# Autodesk Inventor assembly: Galileo Extruder
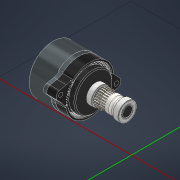
[picture p0: Inventor's stored thumbnail of the model, 180x180]
Saved by Autodesk Inventor 2022.2 (Build 262287010, 287A)
## iProperties
Created: 2022-03-15
Part Number: Galileo Extruder
Document SubType Name: Assembly
Designer: sleib
Author: sleib
## Documents named in this file (7)
- C:\Users\sleib\Projekte\Voron-2\CAD\Inventor\Galileo Clockwork\Galileo Extruder.iam
- C:\Users\sleib\Projekte\Voron-2\CAD\Inventor\Galileo Clockwork\Spacer Shim.ipt
- C:\Users\sleib\Projekte\Voron-2\CAD\Inventor\Galileo Clockwork\Updated Gearset MJF Shaft + Carrier.iam
- C:\Users\sleib\Projekte\Voron-2\CAD\Inventor\Galileo Clockwork\MotorGear.ipt
- C:\Users\sleib\Projekte\Voron-2\CAD\Inventor\Galileo Clockwork\Ring Gear Housing.ipt
- C:\Users\sleib\Projekte\Voron-2\CAD\Inventor\Galileo Clockwork\Stepper Body.ipt
- C:\Users\sleib\Projekte\Voron-2\CAD\Inventor\Galileo Clockwork\MR148ZZ v1.iam
## Components (7 placed, 6 different names)
1. Stepper Body:1 — Passend:17, Fluchtend:1, Passend:18, Passend:19, Passend:20, Fluchtend:2, Passend:21
2. Spacer Shim:1 — Passend:3, Passend:16, Passend:24
3. Updated Gearset MJF Shaft + Carrier:1 [sub-assembly] — Passend:3, Passend:15, Passend:20, Fluchtend:2, Passend:22, Passend:23, Fluchtend:3
4. MotorGear:1 — Passend:15, Passend:16, Passend:25
5. Ring Gear Housing:1 — Passend:18, Passend:19, Passend:21
6. MR148ZZ v1:1 [sub-assembly] — Passend:22, Passend:24
7. MR148ZZ v1:2 [sub-assembly] — Passend:23, Passend:25, Fluchtend:3
## Relationships (15: Mate 12, Flush 3)
- Passend:3 [Mate]: Spacer Shim:1 ↔ Updated Gearset MJF Shaft + Carrier:1
- Passend:15 [Mate]: Updated Gearset MJF Shaft + Carrier:1 ↔ MotorGear:1
- Passend:16 [Mate]: Spacer Shim:1 ↔ MotorGear:1
- Passend:17 [Mate]: Stepper Body:1
- Fluchtend:1 [Flush]: Stepper Body:1
- Passend:18 [Mate]: Stepper Body:1 ↔ Ring Gear Housing:1
- Passend:19 [Mate]: Stepper Body:1 ↔ Ring Gear Housing:1
- Passend:20 [Mate]: Stepper Body:1 ↔ Updated Gearset MJF Shaft + Carrier:1
- Fluchtend:2 [Flush]: Stepper Body:1 ↔ Updated Gearset MJF Shaft + Carrier:1
- Passend:21 [Mate]: Stepper Body:1 ↔ Ring Gear Housing:1
- Passend:22 [Mate]: Updated Gearset MJF Shaft + Carrier:1 ↔ MR148ZZ v1:1
- Passend:23 [Mate]: Updated Gearset MJF Shaft + Carrier:1 ↔ MR148ZZ v1:2
- Passend:24 [Mate]: Spacer Shim:1 ↔ MR148ZZ v1:1
- Passend:25 [Mate]: MotorGear:1 ↔ MR148ZZ v1:2
- Fluchtend:3 [Flush]: Updated Gearset MJF Shaft + Carrier:1 ↔ MR148ZZ v1:2
